# Autodesk Inventor assembly: exhaustFilterHousing
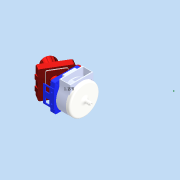
[picture p0: Inventor's stored thumbnail of the model, 180x180]
Saved by Autodesk Inventor 2020 (Build 240168000, 168)
## iProperties
Created: 2020-04-09
Part Number: exhaustFilterHousing
Document SubType Name: Assembly
Designer: Simon
Author: Simon
## Documents named in this file (5)
- D:\GrabCAD\MTL Ventilator Design\Filter housing with o ring\exhaustFilterHousing.iam
- D:\GrabCAD\MTL Ventilator Design\Filter housing with o ring\exhaustboy.ipt
- D:\GrabCAD\MTL Ventilator Design\Filter housing with o ring\check valve v2 v1.ipt
- D:\GrabCAD\MTL Ventilator Design\Filter housing with o ring\exhaustCap.ipt
- D:\GrabCAD\MTL Ventilator Design\Filter housing with o ring\filter_connector v1 (1).ipt
## Components (4 placed, 4 different names)
1. exhaustboy:1 — Mate:1, Mate:2, Angle:1, Mate:3, Mate:4
2. check valve v2 v1:1 — Mate:1, Mate:2, Angle:1, Mate:5, Mate:6
3. exhaustCap:1 — Mate:3, Mate:4
4. filter_connector v1 (1):1 — Mate:5, Mate:6
## Relationships (7: Mate 6, Angle 1)
- Mate:1: exhaustboy:1 ↔ check valve v2 v1:1
- Mate:2: exhaustboy:1 ↔ check valve v2 v1:1
- Angle:1 (0 deg): exhaustboy:1 ↔ check valve v2 v1:1
- Mate:3: exhaustboy:1 ↔ exhaustCap:1
- Mate:4: exhaustboy:1 ↔ exhaustCap:1
- Mate:5: check valve v2 v1:1 ↔ filter_connector v1 (1):1
- Mate:6 (0.25 mm): check valve v2 v1:1 ↔ filter_connector v1 (1):1
